# Autodesk Inventor assembly: FlyCutterSub
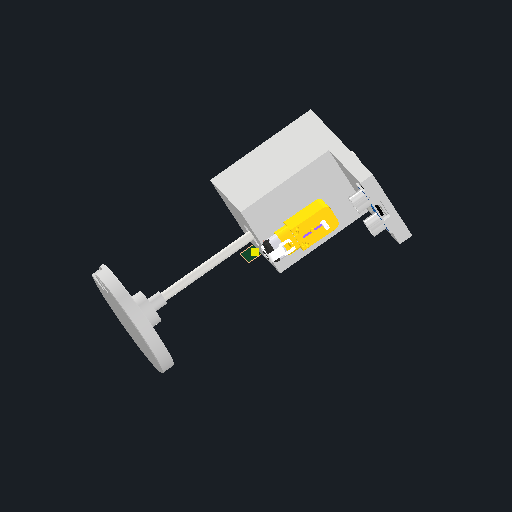
[picture p0: Inventor's stored thumbnail of the model, 512x512]
Saved by Autodesk Inventor 2024.2 (Build 282272000, 272)
## iProperties
Created: 2024-03-19
Part Number: FlyCutterSub
Document SubType Name: Assembly
Designer: LightStore
Author: LightStore
## Documents named in this file (8)
- C:\Users\seifs\Downloads\Final Assembly\FlyCutterSub (1).iam
- C:\Users\seifs\Downloads\Final Assembly\Gearbox.ipt
- C:\Users\seifs\Downloads\Final Assembly\FlyCutter.ipt
- C:\Users\seifs\OneDrive\Documents\Inventor\Content Center Files\R2024\en-US\Bearing GB_T 292-2007\Rolling bearing B708 C GB_T 292-2007.ipt
- C:\Users\seifs\Downloads\Final Assembly\Shaft3.ipt
- C:\Users\seifs\Downloads\Final Assembly\Bevel Gears.iam
- C:\Users\seifs\Downloads\Final Assembly\HC-SR04.ipt
- C:\Users\seifs\Downloads\Final Assembly\Mini Gear DC Motor 6 V Yellow\Mini Gear DC Motor 6 V Yellow.ipt
## Components (8 placed, 7 different names)
1. Gearbox:1 — Insert:11, Insert:12, Insert:16, Mate:2, Insert:18
2. FlyCutter:1 — Insert:19
3. Bearing GB/T 292-2007 Type IN - withdrawn B708 C:1 — Insert:13, Insert:18
4. Bearing GB/T 292-2007 Type IN - withdrawn B708 C:2 — Insert:16
5. Shaft:1 — Insert:13, Mate:1, Insert:19, Mate:3
6. Bevel Gears:1 [sub-assembly] — Insert:14, Mate:1, Mate:2, Mate:3
7. Mini Gear DC Motor 6 V Yellow:1 — Insert:14
8. HC-SR04:1 — Insert:11, Insert:12
## Relationships (10: Insert 7, Mate 3)
- Insert:11: Gearbox:1 ↔ HC-SR04:1
- Insert:12: Gearbox:1 ↔ HC-SR04:1
- Insert:13: Bearing GB/T 292-2007 Type IN - withdrawn B708 C:1 ↔ Shaft:1
- Insert:14: Bevel Gears:1 ↔ Mini Gear DC Motor 6 V Yellow:1
- Insert:16: Gearbox:1 ↔ Bearing GB/T 292-2007 Type IN - withdrawn B708 C:2
- Mate:1: Shaft:1 ↔ Bevel Gears:1
- Mate:2: Gearbox:1 ↔ Bevel Gears:1
- Insert:18: Gearbox:1 ↔ Bearing GB/T 292-2007 Type IN - withdrawn B708 C:1
- Insert:19: FlyCutter:1 ↔ Shaft:1
- Mate:3: Shaft:1 ↔ Bevel Gears:1
